# Autodesk Inventor assembly: ServoMotorsInitialPositioningUnit
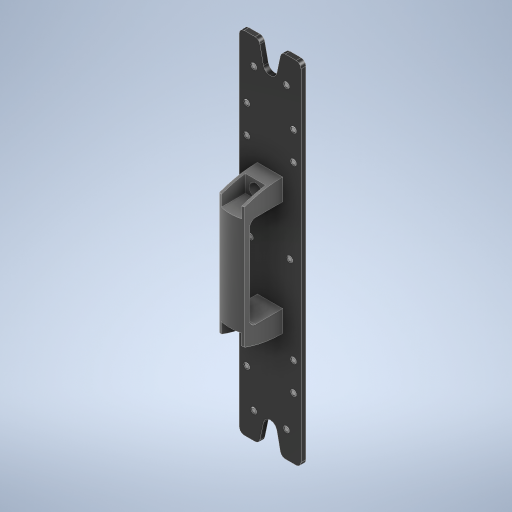
[picture p0: Inventor's stored thumbnail of the model, 512x512]
Saved by Autodesk Inventor 2024.2 (Build 282272000, 272)
## iProperties
Created: 2024-01-11
Part Number: ServoMotorsInitialPositioningUnit
Document SubType Name: Assembly
Designer: Masato Kubotera
Mass: 341.563 g
Surface Area: 687.509 cm^2
Volume: 147.291 cm^3
Density: 2.31896 g/cm^3
Author: Masato Kubotera
## Documents named in this file (4)
- C:\Users\masato\OneDrive - Chiba Institute of Technology\CIT Brains\RoboCup2024\Mechanic\SUSTAINA-OP2\NativeFiles\Boby\OptionComponents\ServoMotorsInitialPositioningUnit.iam
- C:\Users\masato\OneDrive - Chiba Institute of Technology\CIT Brains\RoboCup2024\Mechanic\SUSTAINA-OP2\NativeFiles\Boby\OptionComponents\ServoMotorsInitialPositioningFrame.ipt
- C:\Users\masato\OneDrive - Chiba Institute of Technology\CIT Brains\RoboCup2024\Mechanic\SUSTAINA-OP2\NativeFiles\Boby\COTS\MisumiComponents\SFPSA6-P2-L5-B5.ipt
- C:\Users\masato\OneDrive - Chiba Institute of Technology\CIT Brains\RoboCup2024\Mechanic\SUSTAINA-OP2\NativeFiles\Boby\COTS\MisumiComponents\UPCN26-B-41.ipt
## Components (16 placed, 3 different names)
1. ServoMotorsInitialPositioningFrame:1 — Insert:1, Insert:2, Insert:3, Insert:4, Insert:5, Insert:6, Insert:7, Insert:8, Insert:9, Insert:10, Insert:11, Insert:12, Insert:13, Insert:14, Insert:15
2. SFPSA6-P2-L5-B5:1 — Insert:1
3. SFPSA6-P2-L5-B5:2 — Insert:2
4. SFPSA6-P2-L5-B5:3 — Insert:3
5. SFPSA6-P2-L5-B5:4 — Insert:4
6. SFPSA6-P2-L5-B5:5 — Insert:5
7. SFPSA6-P2-L5-B5:6 — Insert:6
8. SFPSA6-P2-L5-B5:7 — Insert:7
9. SFPSA6-P2-L5-B5:8
10. SFPSA6-P2-L5-B5:9 — Insert:10
11. SFPSA6-P2-L5-B5:10 — Insert:9
12. SFPSA6-P2-L5-B5:11 — Insert:8
13. SFPSA6-P2-L5-B5:12 — Insert:13
14. SFPSA6-P2-L5-B5:13 — Insert:12
15. SFPSA6-P2-L5-B5:14 — Insert:11
16. UPCN26-B-41:1 — Insert:14, Insert:15
## Relationships (15: Insert 15)
- Insert:1: ServoMotorsInitialPositioningFrame:1 ↔ SFPSA6-P2-L5-B5:1
- Insert:2: ServoMotorsInitialPositioningFrame:1 ↔ SFPSA6-P2-L5-B5:2
- Insert:3: ServoMotorsInitialPositioningFrame:1 ↔ SFPSA6-P2-L5-B5:3
- Insert:4: ServoMotorsInitialPositioningFrame:1 ↔ SFPSA6-P2-L5-B5:4
- Insert:5: ServoMotorsInitialPositioningFrame:1 ↔ SFPSA6-P2-L5-B5:5
- Insert:6: ServoMotorsInitialPositioningFrame:1 ↔ SFPSA6-P2-L5-B5:6
- Insert:7: ServoMotorsInitialPositioningFrame:1 ↔ SFPSA6-P2-L5-B5:7
- Insert:8: ServoMotorsInitialPositioningFrame:1 ↔ SFPSA6-P2-L5-B5:11
- Insert:9: ServoMotorsInitialPositioningFrame:1 ↔ SFPSA6-P2-L5-B5:10
- Insert:10: ServoMotorsInitialPositioningFrame:1 ↔ SFPSA6-P2-L5-B5:9
- Insert:11: ServoMotorsInitialPositioningFrame:1 ↔ SFPSA6-P2-L5-B5:14
- Insert:12: ServoMotorsInitialPositioningFrame:1 ↔ SFPSA6-P2-L5-B5:13
- Insert:13: ServoMotorsInitialPositioningFrame:1 ↔ SFPSA6-P2-L5-B5:12
- Insert:14: ServoMotorsInitialPositioningFrame:1 ↔ UPCN26-B-41:1
- Insert:15: ServoMotorsInitialPositioningFrame:1 ↔ UPCN26-B-41:1
